# Autodesk Inventor assembly: COXA_YAW_BLOCK_ASM2
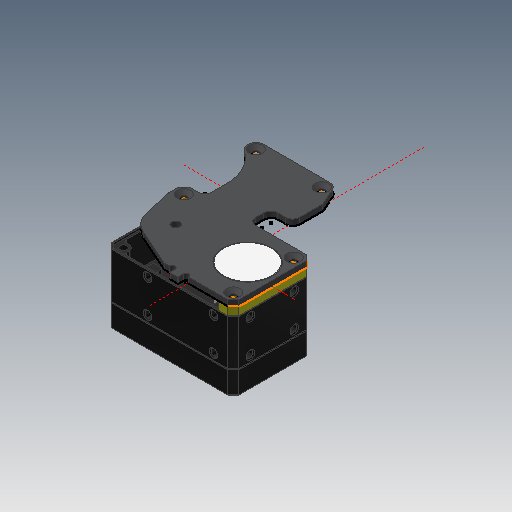
[picture p0: Inventor's stored thumbnail of the model, 512x512]
Saved by Autodesk Inventor 2019.4 (Build 234330000, 330)
## iProperties
Created: 2019-11-06
Part Number: COXA_YAW_BLOCK_ASM2
Material: 一般
Document SubType Name: Assembly
Designer: y6tada
Author: y6tada
## Documents named in this file (4)
- C:\Workspace\Yuni9\Inventor\Asm\COXA_UNIT\COXA_YAW_BLOCK_ASM2.iam
- C:\Workspace\Yuni9\Inventor\Libs\DYNAMIXEL\XM430\XM430_ASM_WITHOUT-BACK.iam
- C:\Workspace\Yuni9\Inventor\Asm\COXA_UNIT\COXA_YAW_ROLL_ADPT_SPACER.ipt
- C:\Workspace\Yuni9\Inventor\Asm\COXA_UNIT\COXA_YAW_ROLL_ADPT_TOP_BASE.ipt
## Components (3 placed, 3 different names)
1. XM430_ASM_WITHOUT-BACK:1 [sub-assembly] — メイト:2
2. COXA_YAW_ROLL_ADPT_SPACER:1 — メイト:2, フラッシュ:2
3. COXA_YAW_ROLL_ADPT_TOP_BASE:1 — フラッシュ:2
## Relationships (5: Mate 3, Flush 2)
- [Flush]: XM430_ASM_WITHOUT-BACK:1 ↔ COXA_YAW_ROLL_ADPT_SPACER:1
- [Mate]: XM430_ASM_WITHOUT-BACK:1 ↔ COXA_YAW_ROLL_ADPT_SPACER:1
- メイト:2 [Mate]: XM430_ASM_WITHOUT-BACK:1 ↔ COXA_YAW_ROLL_ADPT_SPACER:1
- [Mate]: XM430_ASM_WITHOUT-BACK:1 ↔ COXA_YAW_ROLL_ADPT_SPACER:1
- フラッシュ:2 [Flush]: COXA_YAW_ROLL_ADPT_SPACER:1 ↔ COXA_YAW_ROLL_ADPT_TOP_BASE:1
